# Autodesk Inventor assembly: Assembly1
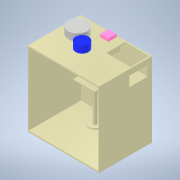
[picture p0: Inventor's stored thumbnail of the model, 180x180]
Saved by Autodesk Inventor 2021 (Build 250183000, 183)
## iProperties
Created: 2022-05-16
Part Number: Assembly1
Document SubType Name: Assembly
Designer: techv
Author: techv
## Documents named in this file (6)
- D:\Projects\P_Baker Bot\Design\Assembly1.iam
- D:\Projects\P_Baker Bot\Design\Outer Casing.ipt
- D:\Projects\P_Baker Bot\Design\Flour Container.ipt
- D:\Projects\P_Baker Bot\Design\water container.ipt
- D:\Projects\P_Baker Bot\Design\oil container.ipt
- D:\Projects\P_Baker Bot\Juicer\mesh body.ipt
## Components (5 placed, 5 different names)
1. Outer Casing:1 — Mate:1, Mate:2, Mate:3, Mate:4, Mate:5, Mate:6, Mate:7
2. Flour Container:1 — Mate:1, Mate:2
3. water container:1 — Mate:3, Mate:4
4. oil container:1 — Mate:5, Mate:6, Mate:7
5. mesh body:1
## Relationships (7: Mate 7)
- Mate:1: Outer Casing:1 ↔ Flour Container:1
- Mate:2: Outer Casing:1 ↔ Flour Container:1
- Mate:3: Outer Casing:1 ↔ water container:1
- Mate:4: Outer Casing:1 ↔ water container:1
- Mate:5: Outer Casing:1 ↔ oil container:1
- Mate:6: Outer Casing:1 ↔ oil container:1
- Mate:7: Outer Casing:1 ↔ oil container:1
